# Autodesk Inventor assembly: Marker Changer - Static Parts
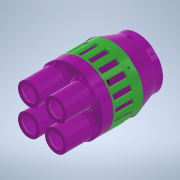
[picture p0: Inventor's stored thumbnail of the model, 180x180]
Saved by Autodesk Inventor 2022.2 (Build 262287000, 287)
## iProperties
Created: 2022-02-09
Part Number: Marker Changer - Static Parts
Document SubType Name: Assembly
Designer: smiku
Author: smiku
## Documents named in this file (6)
- C:\Users\smiku\3D Objects\GrabCAD\AACC Mechatonics Capstone\Marker Changer\Subassemblies\Marker Changer - Static Parts.iam
- C:\Users\smiku\3D Objects\GrabCAD\AACC Mechatonics Capstone\Marker Changer\Cam Barrel Plate.ipt
- C:\Users\smiku\3D Objects\GrabCAD\AACC Mechatonics Capstone\Interface\Servo\DS3225mg Servo.ipt
- C:\Users\smiku\3D Objects\GrabCAD\AACC Mechatonics Capstone\Interface\Interface Block.ipt
- C:\Users\smiku\3D Objects\GrabCAD\AACC Mechatonics Capstone\Marker Changer\Case.ipt
- C:\Users\smiku\3D Objects\GrabCAD\AACC Mechatonics Capstone\Marker Changer\Hoop.ipt
## Components (5 placed, 5 different names)
1. Interface Block:1 — Rigid:7
2. Case:1 — Rigid:6, Rigid:7, Rigid:8
3. DS3225mg Servo:1 — Rigid:6
4. Hoop:1 — Rigid:5, Rigid:8
5. Cam Barrel Plate:1 — Rigid:5
## Relationships (4: WeldJoint 4)
- Rigid:5 [WeldJoint]: Hoop:1 ↔ Cam Barrel Plate:1
- Rigid:6 [WeldJoint]: Case:1 ↔ DS3225mg Servo:1
- Rigid:7 [WeldJoint]: Interface Block:1 ↔ Case:1
- Rigid:8 [WeldJoint]: Case:1 ↔ Hoop:1
